# Autodesk Inventor assembly: Kitchen.00
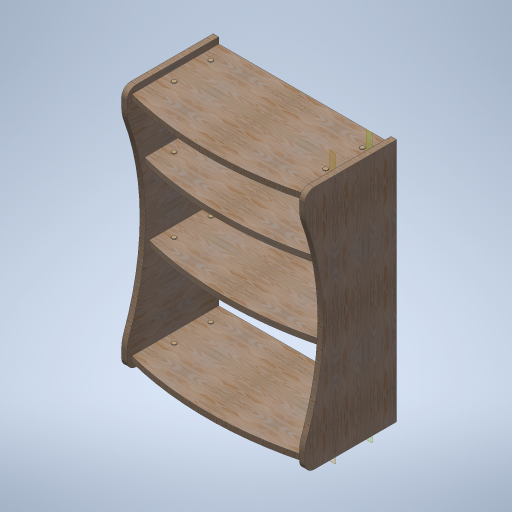
[picture p0: Inventor's stored thumbnail of the model, 512x512]
Saved by Autodesk Inventor 2024 (Build 280153000, 153)
## iProperties
Created: 2016-08-19
Part Number: Kitchen.00
Document SubType Name: Assembly
Designer: SauliusD
Description: Shelf
Author: SauliusD
## Documents named in this file (10)
- C:\W4INV 2024 Design\PROJECTS\Samples\Simple Kitchen table and stool\Shelf\Shelf.iam
- C:\W4INV 2024 Design\PROJECTS\Samples\Simple Kitchen table and stool\Shelf\Top.ipt
- C:\W4INV 2024 Design\PROJECTS\Samples\Simple Kitchen table and stool\Shelf\Shelf 1.ipt
- C:\W4INV 2024 Design\PROJECTS\Samples\Simple Kitchen table and stool\Shelf\Bottom.ipt
- C:\W4INV 2024 Design\PROJECTS\Samples\Simple Kitchen table and stool\Shelf\Shelf 2.ipt
- C:\W4INV 2024 Design\PROJECTS\Samples\Simple Kitchen table and stool\Shelf\Right Side.ipt
- C:\W4INV 2024 Design\PROJECTS\Samples\Simple Kitchen table and stool\Shelf\Left Side.ipt
- C:\W4INV 2024 Design\_LIBRARY\Fixed joints\Minifix joint\MINIFIX D15 v2\Minifix D15 & Dowel L34 & Cap D15 PB T18 LH.ipt
- C:\W4INV 2024 Design\_LIBRARY\Fixed joints\Minifix joint\MINIFIX D15 v2\Minifix D15 & Dowel L34 & Cap D15 PB T18 RH.ipt
- C:\W4INV 2022 Design\LIBRARY\Fixed joints\Minifix joint\MINIFIX D15 v2.ipt
## Components (22 placed, 8 different names)
1. Top:1 — Pillar Board Side Plane :1, Pillar Board Side Plane :2, Pillar Board Side Plane :9, Pillar Board Side Plane :10
2. Shelf 1:1 — Pillar Board Side Plane :3, Pillar Board Side Plane :4, Pillar Board Side Plane :11, Pillar Board Side Plane :12
3. Bottom:1 — Pillar Board Side Plane :7, Pillar Board Side Plane :8, Pillar Board Side Plane :15, Pillar Board Side Plane :16
4. Shelf 2:1 — Pillar Board Side Plane :5, Pillar Board Side Plane :6, Pillar Board Side Plane :13, Pillar Board Side Plane :14
5. Right Side:1 — Flush:1, Flush:2, Nestled Board Plane:2, Nestled Board Plane:4, Nestled Board Plane:6, Nestled Board Plane:8, Nestled Board Plane:10, Nestled Board Plane:12, Nestled Board Plane:14, Nestled Board Plane:16
6. Left Side:1 — Nestled Board Plane:1, Nestled Board Plane:3, Nestled Board Plane:5, Nestled Board Plane:7, Nestled Board Plane:9, Nestled Board Plane:11, Nestled Board Plane:13, Nestled Board Plane:15
7. Minifix D15 & Dowel L34 & Cap D15 PB T18 LH:1 — Axis Plane:1, Pillar Board Side Plane :1, Nestled Board Plane:1
8. Minifix D15 & Dowel L34 & Cap D15 PB T18 RH:2 — Axis Plane:2, Pillar Board Side Plane :2, Nestled Board Plane:2
9. Minifix D15 & Dowel L34 & Cap D15 PB T18 LH:3 — Axis Plane:3, Pillar Board Side Plane :3, Nestled Board Plane:3
10. Minifix D15 & Dowel L34 & Cap D15 PB T18 RH:4 — Axis Plane:4, Pillar Board Side Plane :4, Nestled Board Plane:4
11. Minifix D15 & Dowel L34 & Cap D15 PB T18 LH:5 — Axis Plane:5, Pillar Board Side Plane :5, Nestled Board Plane:5
12. Minifix D15 & Dowel L34 & Cap D15 PB T18 RH:6 — Axis Plane:6, Pillar Board Side Plane :6, Nestled Board Plane:6
13. Minifix D15 & Dowel L34 & Cap D15 PB T18 LH:7 — Axis Plane:7, Pillar Board Side Plane :7, Nestled Board Plane:7
14. Minifix D15 & Dowel L34 & Cap D15 PB T18 RH:8 — Axis Plane:8, Pillar Board Side Plane :8, Nestled Board Plane:8
15. Minifix D15 & Dowel L34 & Cap D15 PB T18 RH:9 — Axis Plane:9, Pillar Board Side Plane :9, Nestled Board Plane:9
16. Minifix D15 & Dowel L34 & Cap D15 PB T18 LH:10 — Axis Plane:10, Pillar Board Side Plane :10, Nestled Board Plane:10
17. Minifix D15 & Dowel L34 & Cap D15 PB T18 RH:11 — Axis Plane:11, Pillar Board Side Plane :11, Nestled Board Plane:11
18. Minifix D15 & Dowel L34 & Cap D15 PB T18 LH:12 — Axis Plane:12, Pillar Board Side Plane :12, Nestled Board Plane:12
19. Minifix D15 & Dowel L34 & Cap D15 PB T18 RH:13 — Axis Plane:13, Pillar Board Side Plane :13, Nestled Board Plane:13
20. Minifix D15 & Dowel L34 & Cap D15 PB T18 LH:14 — Axis Plane:14, Pillar Board Side Plane :14, Nestled Board Plane:14
21. Minifix D15 & Dowel L34 & Cap D15 PB T18 RH:15 — Axis Plane:15, Pillar Board Side Plane :15, Nestled Board Plane:15
22. Minifix D15 & Dowel L34 & Cap D15 PB T18 LH:16 — Axis Plane:16, Pillar Board Side Plane :16, Nestled Board Plane:16
## Relationships (50: Mate 32, Flush 18)
- Flush:1 (-60 mm): Right Side:1
- Flush:2 (-120 mm): Right Side:1
- Axis Plane:1 [Mate]: Minifix D15 & Dowel L34 & Cap D15 PB T18 LH:1
- Pillar Board Side Plane :1 [Flush] (18 mm): Top:1 ↔ Minifix D15 & Dowel L34 & Cap D15 PB T18 LH:1
- Nestled Board Plane:1 [Mate]: Left Side:1 ↔ Minifix D15 & Dowel L34 & Cap D15 PB T18 LH:1
- Axis Plane:2 [Mate]: Minifix D15 & Dowel L34 & Cap D15 PB T18 RH:2
- Pillar Board Side Plane :2 [Flush] (18 mm): Top:1 ↔ Minifix D15 & Dowel L34 & Cap D15 PB T18 RH:2
- Nestled Board Plane:2 [Mate]: Right Side:1 ↔ Minifix D15 & Dowel L34 & Cap D15 PB T18 RH:2
- Axis Plane:3 [Mate]: Minifix D15 & Dowel L34 & Cap D15 PB T18 LH:3
- Pillar Board Side Plane :3 [Flush] (18 mm): Shelf 1:1 ↔ Minifix D15 & Dowel L34 & Cap D15 PB T18 LH:3
- Nestled Board Plane:3 [Mate]: Left Side:1 ↔ Minifix D15 & Dowel L34 & Cap D15 PB T18 LH:3
- Axis Plane:4 [Mate]: Minifix D15 & Dowel L34 & Cap D15 PB T18 RH:4
- Pillar Board Side Plane :4 [Flush] (18 mm): Shelf 1:1 ↔ Minifix D15 & Dowel L34 & Cap D15 PB T18 RH:4
- Nestled Board Plane:4 [Mate]: Right Side:1 ↔ Minifix D15 & Dowel L34 & Cap D15 PB T18 RH:4
- Axis Plane:5 [Mate]: Minifix D15 & Dowel L34 & Cap D15 PB T18 LH:5
- Pillar Board Side Plane :5 [Flush] (18 mm): Shelf 2:1 ↔ Minifix D15 & Dowel L34 & Cap D15 PB T18 LH:5
- Nestled Board Plane:5 [Mate]: Left Side:1 ↔ Minifix D15 & Dowel L34 & Cap D15 PB T18 LH:5
- Axis Plane:6 [Mate]: Minifix D15 & Dowel L34 & Cap D15 PB T18 RH:6
- Pillar Board Side Plane :6 [Flush] (18 mm): Shelf 2:1 ↔ Minifix D15 & Dowel L34 & Cap D15 PB T18 RH:6
- Nestled Board Plane:6 [Mate]: Right Side:1 ↔ Minifix D15 & Dowel L34 & Cap D15 PB T18 RH:6
- Axis Plane:7 [Mate]: Minifix D15 & Dowel L34 & Cap D15 PB T18 LH:7
- Pillar Board Side Plane :7 [Flush] (18 mm): Bottom:1 ↔ Minifix D15 & Dowel L34 & Cap D15 PB T18 LH:7
- Nestled Board Plane:7 [Mate]: Left Side:1 ↔ Minifix D15 & Dowel L34 & Cap D15 PB T18 LH:7
- Axis Plane:8 [Mate]: Minifix D15 & Dowel L34 & Cap D15 PB T18 RH:8
- Pillar Board Side Plane :8 [Flush] (18 mm): Bottom:1 ↔ Minifix D15 & Dowel L34 & Cap D15 PB T18 RH:8
- Nestled Board Plane:8 [Mate]: Right Side:1 ↔ Minifix D15 & Dowel L34 & Cap D15 PB T18 RH:8
- Axis Plane:9 [Mate]: Minifix D15 & Dowel L34 & Cap D15 PB T18 RH:9
- Pillar Board Side Plane :9 [Flush] (18 mm): Top:1 ↔ Minifix D15 & Dowel L34 & Cap D15 PB T18 RH:9
- Nestled Board Plane:9 [Mate]: Left Side:1 ↔ Minifix D15 & Dowel L34 & Cap D15 PB T18 RH:9
- Axis Plane:10 [Mate]: Minifix D15 & Dowel L34 & Cap D15 PB T18 LH:10
- Pillar Board Side Plane :10 [Flush] (18 mm): Top:1 ↔ Minifix D15 & Dowel L34 & Cap D15 PB T18 LH:10
- Nestled Board Plane:10 [Mate]: Right Side:1 ↔ Minifix D15 & Dowel L34 & Cap D15 PB T18 LH:10
- Axis Plane:11 [Mate]: Minifix D15 & Dowel L34 & Cap D15 PB T18 RH:11
- Pillar Board Side Plane :11 [Flush] (18 mm): Shelf 1:1 ↔ Minifix D15 & Dowel L34 & Cap D15 PB T18 RH:11
- Nestled Board Plane:11 [Mate]: Left Side:1 ↔ Minifix D15 & Dowel L34 & Cap D15 PB T18 RH:11
- Axis Plane:12 [Mate]: Minifix D15 & Dowel L34 & Cap D15 PB T18 LH:12
- Pillar Board Side Plane :12 [Flush] (18 mm): Shelf 1:1 ↔ Minifix D15 & Dowel L34 & Cap D15 PB T18 LH:12
- Nestled Board Plane:12 [Mate]: Right Side:1 ↔ Minifix D15 & Dowel L34 & Cap D15 PB T18 LH:12
- Axis Plane:13 [Mate]: Minifix D15 & Dowel L34 & Cap D15 PB T18 RH:13
- Pillar Board Side Plane :13 [Flush] (18 mm): Shelf 2:1 ↔ Minifix D15 & Dowel L34 & Cap D15 PB T18 RH:13
- Nestled Board Plane:13 [Mate]: Left Side:1 ↔ Minifix D15 & Dowel L34 & Cap D15 PB T18 RH:13
- Axis Plane:14 [Mate]: Minifix D15 & Dowel L34 & Cap D15 PB T18 LH:14
- Pillar Board Side Plane :14 [Flush] (18 mm): Shelf 2:1 ↔ Minifix D15 & Dowel L34 & Cap D15 PB T18 LH:14
- Nestled Board Plane:14 [Mate]: Right Side:1 ↔ Minifix D15 & Dowel L34 & Cap D15 PB T18 LH:14
- Axis Plane:15 [Mate]: Minifix D15 & Dowel L34 & Cap D15 PB T18 RH:15
- Pillar Board Side Plane :15 [Flush] (18 mm): Bottom:1 ↔ Minifix D15 & Dowel L34 & Cap D15 PB T18 RH:15
- Nestled Board Plane:15 [Mate]: Left Side:1 ↔ Minifix D15 & Dowel L34 & Cap D15 PB T18 RH:15
- Axis Plane:16 [Mate]: Minifix D15 & Dowel L34 & Cap D15 PB T18 LH:16
- Pillar Board Side Plane :16 [Flush] (18 mm): Bottom:1 ↔ Minifix D15 & Dowel L34 & Cap D15 PB T18 LH:16
- Nestled Board Plane:16 [Mate]: Right Side:1 ↔ Minifix D15 & Dowel L34 & Cap D15 PB T18 LH:16
